# Autodesk Inventor assembly: jubilee_xy_frame_assembly
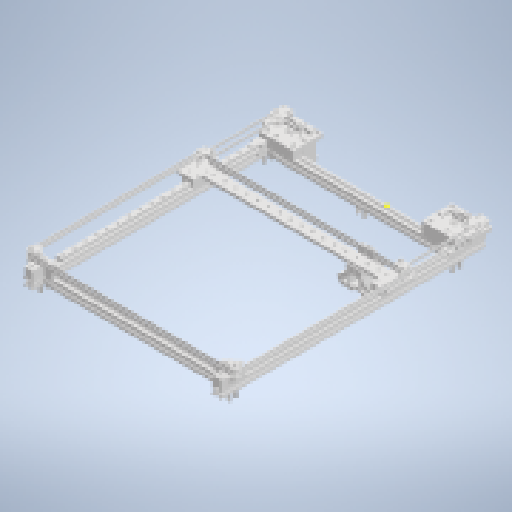
[picture p0: Inventor's stored thumbnail of the model, 512x512]
Saved by Autodesk Inventor 2024.2 (Build 282272000, 272)
## iProperties
Created: 2020-03-16
Part Number: jubilee_xy_frame_assembly
Document SubType Name: Assembly
Designer: Micha
Author: Micha
Revision Number: ANY
## Documents named in this file (13)
- C:\Users\Micha\Documents\493\claw\cad\Inventor\jubilee_xy_frame_assembly.iam
- C:\Users\Micha\Documents\493\claw\cad\Inventor\corexy_frame_assembly.iam
- C:\Users\Micha\Documents\493\claw\cad\Inventor\left_corner_pulley_assembly.iam
- C:\Users\Micha\Documents\493\claw\cad\Inventor\right_corner_pulley_assembly.iam
- C:\Users\Micha\Documents\493\claw\cad\Inventor\left_motor_plate_assembly.iam
- C:\Users\Micha\Documents\493\claw\cad\Inventor\right_motor_plate_assembly.iam
- C:\Users\Micha\Documents\493\claw\cad\Inventor\y_rail_assembly.iam
- C:\Users\Micha\Documents\493\claw\cad\Inventor\y_rail_assembly_1.iam
- C:\Users\Micha\Documents\493\claw\cad\Inventor\m3_10mm_buttonhead_screw_92095A182_92095A182.ipt
- C:\Users\Micha\Documents\493\claw\cad\Inventor\crossbar_with_carriage_center.iam
- C:\Users\Micha\Documents\493\claw\cad\Inventor\back_plate_assembly.iam
- C:\Users\Micha\Documents\493\claw\cad\Inventor\actually_upper_belt.ipt
- C:\Users\Micha\Documents\493\claw\cad\Inventor\actually_lower_belt.ipt
## Components (21 placed, 21 different names)
1. corexy_frame_assembly_283 [sub-assembly] — Flush:1, Flush:2, Flush:3, Flush:4, Mate:1, Flush:5, Flush:6, Mate:2, Mate:3, Flush:7, Flush:8, Mate:4, Flush:9, Mate:5
2. left_corner_pulley_assembly_284 [sub-assembly] — Flush:5, Flush:6, Mate:2
3. right_corner_pulley_assembly_285 [sub-assembly] — Flush:3, Flush:4, Mate:1
4. left_motor_plate_assembly_286 [sub-assembly] — Mate:3, Flush:7, Flush:8, Mate:6
5. right_motor_plate_assembly_287 [sub-assembly] — Flush:1, Flush:2, Mate:4
6. y_rail_assembly_288 [sub-assembly] — Flush:9, Mate:5, Mate:6
7. y_rail_assembly_289 [sub-assembly]
8. m3_10mm_buttonhead_screw_92095A182_92095A182_290
9. m3_10mm_buttonhead_screw_92095A182_92095A182_291
10. m3_10mm_buttonhead_screw_92095A182_92095A182_292
11. m3_10mm_buttonhead_screw_92095A182_92095A182_293
12. m3_10mm_buttonhead_screw_92095A182_92095A182_294
13. m3_10mm_buttonhead_screw_92095A182_92095A182_295
14. m3_10mm_buttonhead_screw_92095A182_92095A182_296
15. m3_10mm_buttonhead_screw_92095A182_92095A182_297
16. crossbar_with_carriage_center_298 [sub-assembly]
17. back_plate_assembly_302 [sub-assembly]
18. m3_10mm_buttonhead_screw_92095A182_92095A182_310
19. m3_10mm_buttonhead_screw_92095A182_92095A182_311
20. actually_upper_belt_314
21. actually_lower_belt_315
## Relationships (15: Flush 9, Mate 6)
- Flush:1: corexy_frame_assembly_283 ↔ right_motor_plate_assembly_287
- Flush:2: corexy_frame_assembly_283 ↔ right_motor_plate_assembly_287
- Flush:3: corexy_frame_assembly_283 ↔ right_corner_pulley_assembly_285
- Flush:4: corexy_frame_assembly_283 ↔ right_corner_pulley_assembly_285
- Mate:1: corexy_frame_assembly_283 ↔ right_corner_pulley_assembly_285
- Flush:5: corexy_frame_assembly_283 ↔ left_corner_pulley_assembly_284
- Flush:6: corexy_frame_assembly_283 ↔ left_corner_pulley_assembly_284
- Mate:2: corexy_frame_assembly_283 ↔ left_corner_pulley_assembly_284
- Mate:3: corexy_frame_assembly_283 ↔ left_motor_plate_assembly_286
- Flush:7: corexy_frame_assembly_283 ↔ left_motor_plate_assembly_286
- Flush:8: corexy_frame_assembly_283 ↔ left_motor_plate_assembly_286
- Mate:4: corexy_frame_assembly_283 ↔ right_motor_plate_assembly_287
- Flush:9 (4 mm): corexy_frame_assembly_283 ↔ y_rail_assembly_288
- Mate:5: corexy_frame_assembly_283 ↔ y_rail_assembly_288
- Mate:6: left_motor_plate_assembly_286 ↔ y_rail_assembly_288
